# Autodesk Inventor assembly: 20220523_Base Servo v13
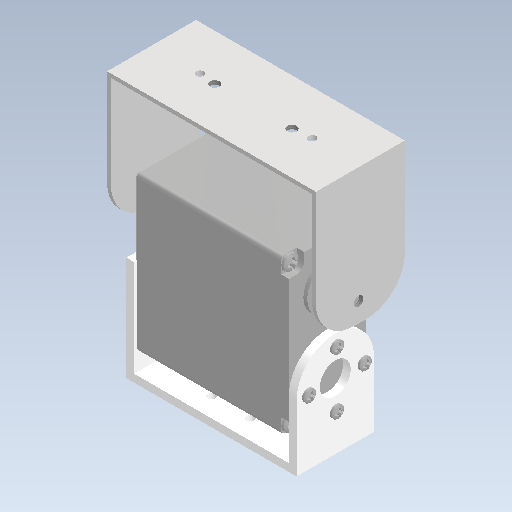
[picture p0: Inventor's stored thumbnail of the model, 512x512]
Saved by Autodesk Inventor 2020 (Build 240168000, 168)
## iProperties
Created: 2022-05-13
Part Number: 20220523_Base Servo v13
Document SubType Name: Assembly
Designer: Naggy
Sending System: Autodesk Translation Framework v10.14.0.1471
Preprocessor: ST-DEVELOPER v18.1
Title: C:/Users/ryusei/Documents/千葉工業大学/Inventor/robot_design4/部品置き場/Base Servo v13.step
## Documents named in this file (5)
- C:\Users\Naggy\Documents\Inventor\robot_design2020\20220523_Base Servo v13.iam
- C:\Users\Naggy\Documents\Inventor\robot_design2020\Bottom bracket.ipt
- C:\Users\Naggy\Documents\Inventor\robot_design2020\Servo.iam
- C:\Users\Naggy\Documents\Inventor\robot_design2020\Screws (1).iam
- C:\Users\Naggy\Documents\Inventor\robot_design2020\20220523_servo_iron.0001.ipt
## Components (4 placed, 4 different names)
1. Bottom bracket:1
2. Servo:1 [sub-assembly] — 挿入:1
3. Screws (1):1 [sub-assembly]
4. 20220523_servo_iron.0001:1 — 挿入:1
## Relationships (1: Insert 1)
- 挿入:1 [Insert] (1 mm): Servo:1 ↔ 20220523_servo_iron.0001:1
